# Autodesk Inventor assembly: proj
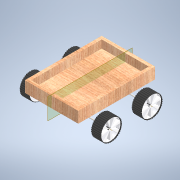
[picture p0: Inventor's stored thumbnail of the model, 180x180]
Saved by Autodesk Inventor 2020 (Build 240168000, 168)
## iProperties
Created: 2020-03-24
Part Number: proj
Document SubType Name: Assembly
Designer: Manish
Author: Manish
## Documents named in this file (6)
- C:\Users\Manish\Documents\inventorassembly\proj.iam
- C:\Users\Manish\Documents\inventorparts\Part1proj.ipt
- C:\Users\Manish\Documents\inventorparts\Part2proj.ipt
- C:\Users\Manish\Documents\inventorassembly\Shaft1.ipt
- C:\Users\Manish\Documents\inventorparts\Part2proj_MIR.ipt
- C:\Users\Manish\Documents\inventorassembly\Shaft1_MIR.ipt
## Components (9 placed, 5 different names)
1. Part1proj:1 — Angle:1, Flush:3
2. Part2proj:1 — Mate:1, Flush:1
3. Shaft:1 — Mate:1, Flush:1, Angle:1
4. Part2proj:2
5. Shaft:2
6. Part2proj_MIR:1 — Mate:3, Mate:4
7. Shaft1_MIR:1 — Mate:3, Mate:4
8. Part2proj_MIR:2 — Mate:5, Mate:6
9. Shaft1_MIR:2 — Mate:5, Mate:6
## Relationships (10: Mate 6, Flush 3, Angle 1)
- Mate:1: Part2proj:1 ↔ Shaft:1
- Flush:1: Part2proj:1 ↔ Shaft:1
- Angle:1 (0 deg): Part1proj:1 ↔ Shaft:1
- [Mate]: Part2proj:2 ↔ Shaft:2
- [Flush]: Part2proj:2 ↔ Shaft:2
- Flush:3 (-125 mm): Part1proj:1
- Mate:3: Part2proj_MIR:1 ↔ Shaft1_MIR:1
- Mate:4: Part2proj_MIR:1 ↔ Shaft1_MIR:1
- Mate:5: Part2proj_MIR:2 ↔ Shaft1_MIR:2
- Mate:6: Part2proj_MIR:2 ↔ Shaft1_MIR:2
## Named parameters: d3_d0 = 0 mm, d4_d1 = 0 mm
